# Autodesk Inventor assembly: jigForHexBushing
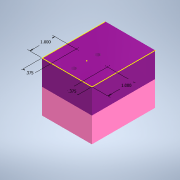
[picture p0: Inventor's stored thumbnail of the model, 180x180]
Saved by Autodesk Inventor 2022.1 (Build 261234000, 234)
## iProperties
Created: 2021-07-26
Part Number: jigForHexBushing
Document SubType Name: Assembly
Designer: robst
Author: robst
## Documents named in this file (3)
- C:\git\CAD-Development\robSteele\ShapeWays\TelescopeProjects\TelescopeMountNov2020\jigForHexBushing.iam
- C:\git\CAD-Development\robSteele\ShapeWays\TelescopeProjects\TelescopeMountNov2020\jigForHexBushingForConnectorPieceBottom.ipt
- C:\git\CAD-Development\robSteele\ShapeWays\TelescopeProjects\TelescopeMountNov2020\jigForHexBushingForConnectorPieceTop.ipt
## Components (2 placed, 2 different names)
1. jigForHexBushingForConnectorPieceBottom:1 — Mate:1, Flush:1, Flush:2
2. jigForHexBushingForConnectorPieceTop:1 — Mate:1, Flush:1, Flush:2
## Relationships (3: Flush 2, Mate 1)
- Mate:1: jigForHexBushingForConnectorPieceBottom:1 ↔ jigForHexBushingForConnectorPieceTop:1
- Flush:1: jigForHexBushingForConnectorPieceBottom:1 ↔ jigForHexBushingForConnectorPieceTop:1
- Flush:2: jigForHexBushingForConnectorPieceBottom:1 ↔ jigForHexBushingForConnectorPieceTop:1
